# Autodesk Inventor assembly: handle_base
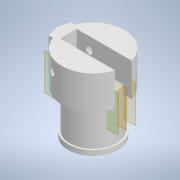
[picture p0: Inventor's stored thumbnail of the model, 180x180]
Saved by Autodesk Inventor 2022 (Build 260153000, 153)
## iProperties
Created: 2021-08-15
Part Number: handle_base
Document SubType Name: Assembly
Designer: teh18
Author: teh18
## Documents named in this file (3)
- C:\Users\ben\Documents\GitHub\r68-bve-mascon\handle-base\handle_base.iam
- C:\Users\ben\Documents\GitHub\r68-bve-mascon\handle-base\top.ipt
- C:\Users\ben\Documents\GitHub\r68-bve-mascon\handle-base\bottom.ipt
## Components (2 placed, 2 different names)
1. top:1
2. bottom:1
## Relationships (1: Symmetry 1)
- Symmetry:1
